# Autodesk Inventor assembly: Molde_resina_stock_aluminio
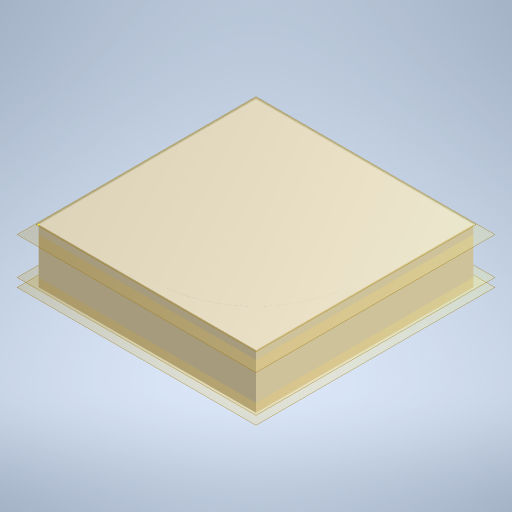
[picture p0: Inventor's stored thumbnail of the model, 512x512]
Saved by Autodesk Inventor 2023.2 (Build 272271030, 271C)
## iProperties
Created: 2023-07-31
Part Number: Molde_resina_stock_aluminio
Document SubType Name: Assembly
Designer: Cris Pat
Author: Cris Pat
## Documents named in this file (3)
- C:\Users\Cris Pat\Desktop\U\Semestre_10\Disenio_y_manufactura\proyecto\Molde_resina_stock_aluminio.iam
- C:\Users\Cris Pat\Desktop\U\Semestre_10\Disenio_y_manufactura\proyecto\molde_resina.ipt
- C:\Users\Cris Pat\Desktop\U\Semestre_10\Disenio_y_manufactura\proyecto\stock_aluminio.ipt
## Components (2 placed, 2 different names)
1. molde_resina:1
2. stock_aluminio:1 — Flush:1, Flush:2
## Relationships (2: Flush 2)
- Flush:1: stock_aluminio:1
- Flush:2: stock_aluminio:1
